# Autodesk Inventor assembly: adjustable_rod
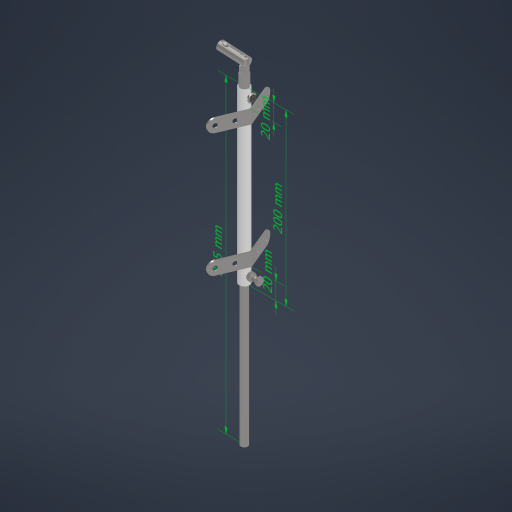
[picture p0: Inventor's stored thumbnail of the model, 512x512]
Saved by Autodesk Inventor 2023 (Build 270158000, 158)
## iProperties
Created: 2022-04-25
Part Number: adjustable_rod
Document SubType Name: Assembly
Designer: Norbert Ligas
Mass: 170.803 g
Surface Area: 276.995 cm^2
Volume: 25.9266 cm^3
Density: 6.58796 g/cm^3
leg_min_length: 200,000 mm
leg_max_length: 365,000 mm
iron_angle_to_pipe_edge: 20,000 mm
pipe_length: 200,000 mm
Author: Norbert Ligas
## Documents named in this file (9)
- C:\Users\norbe\Repozytoria\NormalMapScanner\stand_construction\parts\adjustable_leg.iam
- C:\Users\norbe\Repozytoria\NormalMapScanner\stand_construction\parts\bar_185mm.ipt
- C:\Users\norbe\Repozytoria\NormalMapScanner\stand_construction\parts\pipe_200mm.ipt
- C:\Users\norbe\OneDrive\Dokumenty\Inventor\Content Center Files\R2023\en-US\ISO 4032(2)\ISO 4032 - M5 - ISO.ipt
- C:\Users\norbe\Repozytoria\NormalMapScanner\stand_construction\parts\barrel_hinge.iam
- C:\Users\norbe\OneDrive\Dokumenty\Inventor\Content Center Files\R2023\en-US\ISO 4017(1)\ISO 4017 - M5 x 16 - ISO.ipt
- C:\Users\norbe\OneDrive\Dokumenty\Inventor\Content Center Files\R2023\en-US\ISO 7045  Z\ISO 7045 - M3,5 x 14_ - 4.8 - Z - ISO.ipt
- C:\Users\norbe\OneDrive\Dokumenty\Inventor\Content Center Files\R2023\en-US\ISO 7090\ISO 7090 - 5 - 140 HV(1).ipt
- C:\Users\norbe\Repozytoria\NormalMapScanner\stand_construction\parts\angle_iron.ipt
## Components (9 placed, 8 different names)
1. bar_185mm:1 — Mate:1, Mate:2, Mate:3, Cylindrical:1
2. pipe_200mm:1 — Cylindrical:1, Tangent:1, Mate:5, Mate:7, Mate:8, Angle:4, Mate:10, Mate:11, Tangent:2, Tangent:3, Tangent:4, Mate:12, Tangent:5, Tangent:6, Mate:13, Mate:14, Flush:2
3. ISO 4032 M5:1 — Tangent:1, Mate:5, Mate:10, Insert:1
4. barrel_hinge:1 [sub-assembly] — Mate:7, Mate:8, Mate:11, Insert:2, Mate:14
5. ISO 4017 M5 x 16:1 — Insert:1
6. ISO 7045 Z M3,5 x 14 - 4.8 - Z:1 — Insert:2, Insert:3
7. ISO 7090 5 - 140 HV:1 — Insert:3
8. angle_iron:1 — Tangent:2, Tangent:5, Tangent:6, Mate:13, Flush:1
9. angle_iron:2 — Tangent:3, Tangent:4, Mate:12, Flush:1, Flush:2
## Relationships (24: Mate 11, Tangent 6, Insert 3, Flush 2, CylindricalJoint 1, Angle 1)
- Mate:1: bar_185mm:1
- Mate:2: bar_185mm:1
- Mate:3: bar_185mm:1
- Cylindrical:1: bar_185mm:1 ↔ pipe_200mm:1
- Tangent:1: pipe_200mm:1 ↔ ISO 4032 M5:1
- Mate:5 (10 mm): pipe_200mm:1 ↔ ISO 4032 M5:1
- Mate:7 (-15 mm): pipe_200mm:1 ↔ barrel_hinge:1
- Mate:8: pipe_200mm:1 ↔ barrel_hinge:1
- Angle:4 (0 deg): pipe_200mm:1
- Mate:10: pipe_200mm:1 ↔ ISO 4032 M5:1
- Mate:11: pipe_200mm:1 ↔ barrel_hinge:1
- Insert:1 (5 mm): ISO 4032 M5:1 ↔ ISO 4017 M5 x 16:1
- Insert:2 (7 mm): barrel_hinge:1 ↔ ISO 7045 Z M3,5 x 14 - 4.8 - Z:1
- Insert:3: ISO 7045 Z M3,5 x 14 - 4.8 - Z:1 ↔ ISO 7090 5 - 140 HV:1
- Tangent:2: pipe_200mm:1 ↔ angle_iron:1
- Tangent:3: pipe_200mm:1 ↔ angle_iron:2
- Tangent:4: pipe_200mm:1 ↔ angle_iron:2
- Mate:12 (20 mm): pipe_200mm:1 ↔ angle_iron:2
- Tangent:5: pipe_200mm:1 ↔ angle_iron:1
- Tangent:6: pipe_200mm:1 ↔ angle_iron:1
- Mate:13 (20 mm): pipe_200mm:1 ↔ angle_iron:1
- Mate:14: pipe_200mm:1 ↔ barrel_hinge:1
- Flush:1: angle_iron:1 ↔ angle_iron:2
- Flush:2: pipe_200mm:1 ↔ angle_iron:2
## Named parameters: pipe_length = 200 mm, bar_length = 185 mm, leg_min_length = 200 mm, leg_max_length = 365 mm, max_extrusion = 165 mm, min_extrusion = 0 mm, hinge_insertion = 15 mm, connection_length = 20 mm, current_extrusion = 0 mm, iron_angle_to_pipe_edge = 20 mm
